# Autodesk Inventor assembly: PCBPT_V3
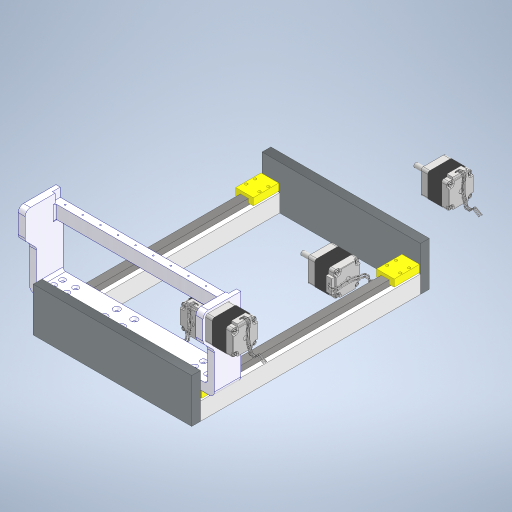
[picture p0: Inventor's stored thumbnail of the model, 512x512]
Saved by Autodesk Inventor 2024 (Build 280153000, 153)
## iProperties
Created: 2023-08-11
Part Number: PCBPT_V3
Document SubType Name: Assembly
Designer: l1534
Author: l1534
## Documents named in this file (7)
- C:\DATA\Documents\Lab\github\PCBPT\PCBPT_V3\Mechanical\PCBPT_V3.iam
- C:\DATA\Documents\Lab\github\PCBPT\PCBPT_V3\Mechanical\wall.ipt
- C:\DATA\Documents\Lab\github\PCBPT\PCBPT_V3\Mechanical\NEMA11\NEMA11.iam
- C:\DATA\Documents\Lab\github\PCBPT\PCBPT_V3\Mechanical\2020x260mm.ipt
- C:\DATA\Documents\Lab\github\PCBPT\PCBPT_V3\Mechanical\MGN9_rail.ipt
- C:\DATA\Documents\Lab\github\PCBPT\PCBPT_V3\Mechanical\MGN9C_block.ipt
- C:\DATA\Documents\Lab\github\PCBPT\PCBPT_V3\Mechanical\gantry_R.ipt
## Components (15 placed, 6 different names)
1. wall:1 — Rigid:1, Rigid:2
2. NEMA11:1 [sub-assembly]
3. 2020x250mm:1 — Rigid:1, Rigid:5
4. 2020x250mm:2 — Rigid:2, Rigid:3, Rigid:4
5. wall:2 — Rigid:3
6. NEMA11:2 [sub-assembly]
7. MGN9_rail:1 — Rigid:4, Slider:2, Slider:3
8. MGN9_rail:2 — Rigid:5, Slider:1, Slider:4
9. MGN9C_block:1 — Slider:4, Flush:2
10. MGN9C_block:2 — Slider:2, Flush:1
11. MGN9C_block:3 — Slider:1, Flush:1, Rigid:8
12. MGN9C_block:4 — Slider:3, Flush:2
13. NEMA11:3 [sub-assembly]
14. NEMA11:4 [sub-assembly] — Insert:1
15. gantry_R:1 — Rigid:8, Insert:1
## Relationships (13: WeldJoint 6, TranslationJoint 4, Flush 2, Insert 1)
- Rigid:1 [WeldJoint]: wall:1 ↔ 2020x250mm:1
- Rigid:2 [WeldJoint]: wall:1 ↔ 2020x250mm:2
- Rigid:3 [WeldJoint]: 2020x250mm:2 ↔ wall:2
- Rigid:4 [WeldJoint]: 2020x250mm:2 ↔ MGN9_rail:1
- Rigid:5 [WeldJoint]: 2020x250mm:1 ↔ MGN9_rail:2
- Slider:1 [TranslationJoint]: MGN9_rail:2 ↔ MGN9C_block:3
- Slider:2 [TranslationJoint]: MGN9_rail:1 ↔ MGN9C_block:2
- Slider:3 [TranslationJoint]: MGN9_rail:1 ↔ MGN9C_block:4
- Slider:4 [TranslationJoint]: MGN9_rail:2 ↔ MGN9C_block:1
- Flush:1: MGN9C_block:2 ↔ MGN9C_block:3
- Flush:2: MGN9C_block:1 ↔ MGN9C_block:4
- Rigid:8 [WeldJoint]: MGN9C_block:3 ↔ gantry_R:1
- Insert:1: NEMA11:4 ↔ gantry_R:1
